# Autodesk Inventor assembly: canon_reservoir
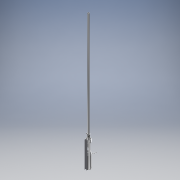
[picture p0: Inventor's stored thumbnail of the model, 180x180]
Saved by Autodesk Inventor 2019 (Build 230136000, 136)
## iProperties
Created: 2019-03-25
Part Number: canon_reservoir
Material: Générique
Document SubType Name: Assembly
Designer: theor
Mass: 835.143 g
Surface Area: 1861.5 cm^2
Volume: 213.821 cm^3
Density: 3.9058 g/cm^3
Author: theor
## Documents named in this file (13)
- C:\dev\projects\ace\ace-git\ACE-FP 12 Prot 2\canon_reservoir.iam
- C:\dev\projects\ace\ace-git\ACE-FP 12 Prot 2\tube_reservoir.ipt
- C:\dev\projects\ace\ace-git\ACE-FP 12 Prot 2\reservoir_jointure.ipt
- C:\dev\projects\ace\ace-git\ACE-FP 12 Prot 2\support_douille.ipt
- C:\dev\projects\ace\ace-git\ACE-FP 12 Prot 2\tube_canon.ipt
- C:\dev\projects\ace\ace-git\ACE-FP 12 Prot 2\piston_reservoir.ipt
- C:\dev\projects\ace\ace-git\ACE-FP 12 Prot 2\support_principal.ipt
- C:\dev\projects\ace\ace-git\ACE-FP 12 Prot 2\support_canon.ipt
- C:\dev\projects\ace\ace-git\ACE-FP 12 Prot 2\douille.ipt
- C:\dev\projects\ace\ace-git\ACE-FP 12 Prot 2\ressort_canon.ipt
- C:\dev\projects\ace\ace-git\ACE-FP 12 Prot 2\blocage_ressort_canon.ipt
- C:\dev\projects\ace\ace-git\ACE-FP 12 Prot 2\support_lateral.ipt
- C:\dev\projects\ace\ace-git\ACE-FP 12 Prot 2\tige_serrage_main.ipt
## Components (13 placed, 12 different names)
1. support_principal:1 — Placage:1, Placage:2, Placage:6, Placage:11, Placage:14
2. piston_reservoir:1 — Placage:1, Placage:2, Placage:3, Placage:19, Placage:20, Placage:22, Placage:23
3. tube_reservoir:1 — Placage:3, Placage:4, Placage:5, Placage:7
4. reservoir_jointure:1 — Placage:5, Placage:6, Placage:7, Placage:8, Placage:25, Placage:26
5. support_douille:1 — Placage:8, Placage:9, Placage:10, Placage:12, Placage:13, Placage:18
6. tube_canon:1 — Placage:9, Placage:10, Placage:15, Placage:16
7. support_canon:1 — Placage:11, Placage:12, Placage:14, Placage:17, Placage:21, Placage:24
8. douille:1 — Placage:13
9. ressort_canon:1 — Placage:15, Placage:17
10. blocage_ressort_canon:1 — Placage:16, Placage:18
11. support_lateral:1 — Placage:19, Placage:20, Placage:21
12. support_lateral:2 — Placage:22, Placage:23, Placage:24
13. tige_serrage_main:1 — Placage:25, Placage:26
## Relationships (26: Mate 26)
- Placage:1 [Mate]: support_principal:1 ↔ piston_reservoir:1
- Placage:2 [Mate]: support_principal:1 ↔ piston_reservoir:1
- Placage:3 [Mate]: piston_reservoir:1 ↔ tube_reservoir:1
- Placage:4 [Mate]: tube_reservoir:1
- Placage:5 [Mate]: tube_reservoir:1 ↔ reservoir_jointure:1
- Placage:6 [Mate]: support_principal:1 ↔ reservoir_jointure:1
- Placage:7 [Mate]: tube_reservoir:1 ↔ reservoir_jointure:1
- Placage:8 [Mate]: reservoir_jointure:1 ↔ support_douille:1
- Placage:9 [Mate]: support_douille:1 ↔ tube_canon:1
- Placage:10 [Mate]: support_douille:1 ↔ tube_canon:1
- Placage:11 [Mate]: support_principal:1 ↔ support_canon:1
- Placage:12 [Mate]: support_douille:1 ↔ support_canon:1
- Placage:13 [Mate]: support_douille:1 ↔ douille:1
- Placage:14 [Mate]: support_principal:1 ↔ support_canon:1
- Placage:15 [Mate]: tube_canon:1 ↔ ressort_canon:1
- Placage:16 [Mate]: tube_canon:1 ↔ blocage_ressort_canon:1
- Placage:17 [Mate]: support_canon:1 ↔ ressort_canon:1
- Placage:18 [Mate] (30 mm): support_douille:1 ↔ blocage_ressort_canon:1
- Placage:19 [Mate]: piston_reservoir:1 ↔ support_lateral:1
- Placage:20 [Mate]: piston_reservoir:1 ↔ support_lateral:1
- Placage:21 [Mate]: support_canon:1 ↔ support_lateral:1
- Placage:22 [Mate]: piston_reservoir:1 ↔ support_lateral:2
- Placage:23 [Mate]: piston_reservoir:1 ↔ support_lateral:2
- Placage:24 [Mate]: support_canon:1 ↔ support_lateral:2
- Placage:25 [Mate]: reservoir_jointure:1 ↔ tige_serrage_main:1
- Placage:26 [Mate]: reservoir_jointure:1 ↔ tige_serrage_main:1
